# Autodesk Inventor assembly: PARA TMP_1L
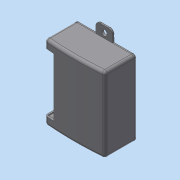
[picture p0: Inventor's stored thumbnail of the model, 180x180]
Saved by Autodesk Inventor 2013 (Build 170138000, 138)
## iProperties
Created: 2018-10-18
Part Number: PARA TMP_1L
Document SubType Name: Assembly
Designer: Fede
Author: Fede
## Documents named in this file (4)
- C:\0000 FEDE\16GB\0000 INTERIOR\PFP_TMP_1L\3d\PARA TMP_1L.iam
- C:\0000 FEDE\16GB\0000 INTERIOR\PFP_TMP_1L\3d\cuerpo.ipt
- C:\0000 FEDE\16GB\0000 INTERIOR\PFP_TMP_1L\3d\tapa.ipt
- C:\0000 FEDE\256GB\inventor\2017-10-23 HORNO CERAMICA\Imported Components\TMP_1L\TMP_1L.iam
## Components (3 placed, 3 different names)
1. cuerpo:1 — Mate:1, Flush:1, Flush:2
2. tapa:1 — Mate:1, Flush:1, Flush:2, Mate:2, Angle:1
3. TMP_1L:1 [sub-assembly] — Mate:2, Angle:1
## Relationships (5: Mate 2, Flush 2, Angle 1)
- Mate:1: cuerpo:1 ↔ tapa:1
- Flush:1: cuerpo:1 ↔ tapa:1
- Flush:2: cuerpo:1 ↔ tapa:1
- Mate:2 (1 mm): tapa:1 ↔ TMP_1L:1
- Angle:1 (0 deg): tapa:1 ↔ TMP_1L:1
